# Autodesk Inventor assembly: Złożenie całości
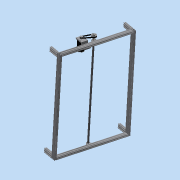
[picture p0: Inventor's stored thumbnail of the model, 180x180]
Saved by Autodesk Inventor 2018 (Build 220112000, 112)
## iProperties
Created: 2019-01-23
Part Number: Złożenie całości
Material: Ogólny
Document SubType Name: Assembly
Designer: Dawid
Author: Dawid
## Documents named in this file (16)
- E:\Frezarka_K2\INVENTOR\ZŁOŻENIA\Złożenie całości.iam
- E:\Frezarka_K2\INVENTOR\RAMA\Profil dolny długi.ipt
- E:\Frezarka_K2\INVENTOR\RAMA\Profil dolny krótki.ipt
- E:\Frezarka_K2\INVENTOR\RAMA\Profil dolny - noga.ipt
- E:\Frezarka_K2\INVENTOR\NAPĘD\Śruba trapezowa 16x4.ipt
- E:\Frezarka_K2\INVENTOR\NAPĘD\Łożysko w obudowie aluminiowej 10mm KP000.ipt
- C:\Users\Dawid\Documents\Inventor\Content Center Files\R2018\pl-PL\DIN 6926\DIN 6926 - M10 x 1,5.ipt
- E:\Frezarka_K2\INVENTOR\NAPĘD\Koło zębate 21 T5 28 2F.ipt
- E:\Frezarka_K2\INVENTOR\NAPĘD\Tuleja zaciskowo rozprężna RCK BK 80 8x15 Clampex.ipt
- C:\Users\Dawid\Documents\Inventor\Content Center Files\R2018\pl-PL\CNS 3932\CNS 3932 - M 4 x 0,7 x 6.ipt
- E:\Frezarka_K2\INVENTOR\NAPĘD\Silnik krokowy SM 60 100-4004AF - 4Nm.ipt
- E:\Frezarka_K2\INVENTOR\NAPĘD\Koło zębate 21 T5 14 2F.ipt
- E:\Frezarka_K2\INVENTOR\NAPĘD\Uchwyt silnika krokowego osi Y.ipt
- C:\Users\Dawid\Documents\Inventor\Content Center Files\R2018\pl-PL\CNS 3932\CNS 3932 - M 5 x 0,8 x 12.ipt
- E:\Frezarka_K2\INVENTOR\NAPĘD\Pas zębaty 10 T5-315.ipt
- C:\Users\Dawid\Documents\Inventor\Content Center Files\R2018\pl-PL\CNS 3932\CNS 3932 - M 5 x 0,8 x 10.ipt
## Components (32 placed, 15 different names)
1. Profil dolny długi:1 — Zestawiający:1, Równoległy:1, Równoległy:2, Zestawiający:4, Równoległy:7, Zestawiający:7, Równoległy:13, Równoległy:14
2. Profil dolny krótki:1 — Zestawiający:1, Równoległy:1, Równoległy:2, Zestawiający:2, Równoległy:3, Równoległy:4, Zestawiający:15
3. Profil dolny długi:2 — Zestawiający:2, Równoległy:3, Równoległy:4, Zestawiający:3, Równoległy:5, Zestawiający:5, Równoległy:9, Równoległy:10, Zestawiający:6, Równoległy:11, Równoległy:12, Równoległy:15, Zestawiający:20
4. Profil dolny krótki:2 — Zestawiający:3, Równoległy:5, Równoległy:8, Równoległy:15, Zestawiający:14, Równoległy:16, Zestawiający:26, Zestawiający:27, Zestawiający:30
5. Profil dolny - noga:1 — Zestawiający:5, Równoległy:9, Równoległy:10
6. Profil dolny - noga:2 — Zestawiający:6, Równoległy:11, Równoległy:12
7. Profil dolny - noga:3 — Zestawiający:7, Równoległy:13, Równoległy:14
8. Profil dolny - noga:4 — Zestawiający:4, Równoległy:7, Równoległy:8
9. Śruba trapezowa 16x4:1 — Zestawiający:8, Zestawiający:9, Zestawiający:10, Zestawiający:11, Zestawiający:12, Zestawiający:18, Zestawiający:19
10. Łożysko w obudowie aluminiowej 10mm KP000:1 — Zestawiający:8, Zestawiający:9, Zestawiający:13, Zestawiający:14, Równoległy:16, Zestawiający:20
11. Łożysko w obudowie aluminiowej 10mm KP000:2 — Zestawiający:10, Zestawiający:11, Zestawiający:15
12. DIN 6926 - zastąpiona przez DIN EN 1663/1666 M10:1 — Zestawiający:12, Zestawiający:13
13. Koło zębate 21 T5 28 2F:1 — Zestawiający:16, Zestawiający:17, Zestawiający:28
14. Tuleja zaciskowo rozprężna RCK BK 80 8x15 Clampex:1 — Zestawiający:16, Zestawiający:17, Zestawiający:18, Zestawiający:19, Wstaw:1, Wstaw:2, Wstaw:3, Wstaw:4, Wstaw:5, Wstaw:6
15. CNS 3932 M 4 x 6:1 — Wstaw:1
16. CNS 3932 M 4 x 6:2 — Wstaw:2
17. CNS 3932 M 4 x 6:3 — Wstaw:3
18. CNS 3932 M 4 x 6:4 — Wstaw:4
19. CNS 3932 M 4 x 6:5 — Wstaw:5
20. CNS 3932 M 4 x 6:6 — Wstaw:6
21. Silnik krokowy SM 60 100-4004AF - 4Nm:1 — Zestawiający:21, Zestawiający:22, Zestawiający:23, Zestawiający:24, Zestawiający:25, Wstaw:7, Wstaw:8, Wstaw:9, Wstaw:10
22. Koło zębate 21 T5 14 2F:1 — Zestawiający:21, Zestawiający:22, Zestawiający:27, Zestawiający:29
23. Uchwyt silnika krokowego osi Y:1 — Zestawiający:23, Zestawiający:24, Zestawiający:25, Zestawiający:26, Zestawiający:30, Wstaw:11, Wstaw:12, Wstaw:13, Wstaw:14
24. CNS 3932 M 5 x 12:1 — Wstaw:7
25. CNS 3932 M 5 x 12:2 — Wstaw:8
26. CNS 3932 M 5 x 12:3 — Wstaw:9
27. CNS 3932 M 5 x 12:4 — Wstaw:10
28. Pas zębaty 10 T5-315:1 — Zestawiający:28, Zestawiający:29
29. CNS 3932 M 5 x 10:1 — Wstaw:11
30. CNS 3932 M 5 x 10:2 — Wstaw:12
31. CNS 3932 M 5 x 10:3 — Wstaw:13
32. CNS 3932 M 5 x 10:4 — Wstaw:14
## Relationships (59: Mate 30, Flush 15, Insert 14)
- Zestawiający:1 [Mate]: Profil dolny długi:1 ↔ Profil dolny krótki:1
- Równoległy:1 [Flush]: Profil dolny długi:1 ↔ Profil dolny krótki:1
- Równoległy:2 [Flush]: Profil dolny długi:1 ↔ Profil dolny krótki:1
- Zestawiający:2 [Mate]: Profil dolny krótki:1 ↔ Profil dolny długi:2
- Równoległy:3 [Flush]: Profil dolny krótki:1 ↔ Profil dolny długi:2
- Równoległy:4 [Flush]: Profil dolny krótki:1 ↔ Profil dolny długi:2
- Zestawiający:3 [Mate]: Profil dolny długi:2 ↔ Profil dolny krótki:2
- Równoległy:5 [Flush]: Profil dolny długi:2 ↔ Profil dolny krótki:2
- Zestawiający:4 [Mate]: Profil dolny długi:1 ↔ Profil dolny - noga:4
- Równoległy:7 [Flush]: Profil dolny długi:1 ↔ Profil dolny - noga:4
- Równoległy:8 [Flush]: Profil dolny krótki:2 ↔ Profil dolny - noga:4
- Zestawiający:5 [Mate]: Profil dolny długi:2 ↔ Profil dolny - noga:1
- Równoległy:9 [Flush]: Profil dolny długi:2 ↔ Profil dolny - noga:1
- Równoległy:10 [Flush]: Profil dolny długi:2 ↔ Profil dolny - noga:1
- Zestawiający:6 [Mate]: Profil dolny długi:2 ↔ Profil dolny - noga:2
- Równoległy:11 [Flush]: Profil dolny długi:2 ↔ Profil dolny - noga:2
- Równoległy:12 [Flush]: Profil dolny długi:2 ↔ Profil dolny - noga:2
- Zestawiający:7 [Mate]: Profil dolny długi:1 ↔ Profil dolny - noga:3
- Równoległy:13 [Flush]: Profil dolny długi:1 ↔ Profil dolny - noga:3
- Równoległy:14 [Flush]: Profil dolny długi:1 ↔ Profil dolny - noga:3
- Zestawiający:8 [Mate]: Śruba trapezowa 16x4:1 ↔ Łożysko w obudowie aluminiowej 10mm KP000:1
- Zestawiający:9 [Mate]: Śruba trapezowa 16x4:1 ↔ Łożysko w obudowie aluminiowej 10mm KP000:1
- Zestawiający:10 [Mate]: Śruba trapezowa 16x4:1 ↔ Łożysko w obudowie aluminiowej 10mm KP000:2
- Zestawiający:11 [Mate] (2 mm): Śruba trapezowa 16x4:1 ↔ Łożysko w obudowie aluminiowej 10mm KP000:2
- Zestawiający:12 [Mate]: Śruba trapezowa 16x4:1 ↔ DIN 6926 - zastąpiona przez DIN EN 1663/1666 M10:1
- Zestawiający:13 [Mate]: Łożysko w obudowie aluminiowej 10mm KP000:1 ↔ DIN 6926 - zastąpiona przez DIN EN 1663/1666 M10:1
- Równoległy:15 [Flush]: Profil dolny długi:2 ↔ Profil dolny krótki:2
- Zestawiający:14 [Mate]: Profil dolny krótki:2 ↔ Łożysko w obudowie aluminiowej 10mm KP000:1
- Równoległy:16 [Flush] (2 mm): Profil dolny krótki:2 ↔ Łożysko w obudowie aluminiowej 10mm KP000:1
- Zestawiający:15 [Mate]: Profil dolny krótki:1 ↔ Łożysko w obudowie aluminiowej 10mm KP000:2
- Zestawiający:16 [Mate]: Koło zębate 21 T5 28 2F:1 ↔ Tuleja zaciskowo rozprężna RCK BK 80 8x15 Clampex:1
- Zestawiający:17 [Mate]: Koło zębate 21 T5 28 2F:1 ↔ Tuleja zaciskowo rozprężna RCK BK 80 8x15 Clampex:1
- Zestawiający:18 [Mate]: Śruba trapezowa 16x4:1 ↔ Tuleja zaciskowo rozprężna RCK BK 80 8x15 Clampex:1
- Zestawiający:19 [Mate] (2 mm): Śruba trapezowa 16x4:1 ↔ Tuleja zaciskowo rozprężna RCK BK 80 8x15 Clampex:1
- Wstaw:1 [Insert]: Tuleja zaciskowo rozprężna RCK BK 80 8x15 Clampex:1 ↔ CNS 3932 M 4 x 6:1
- Wstaw:2 [Insert]: Tuleja zaciskowo rozprężna RCK BK 80 8x15 Clampex:1 ↔ CNS 3932 M 4 x 6:2
- Wstaw:3 [Insert]: Tuleja zaciskowo rozprężna RCK BK 80 8x15 Clampex:1 ↔ CNS 3932 M 4 x 6:3
- Wstaw:4 [Insert]: Tuleja zaciskowo rozprężna RCK BK 80 8x15 Clampex:1 ↔ CNS 3932 M 4 x 6:4
- Wstaw:5 [Insert]: Tuleja zaciskowo rozprężna RCK BK 80 8x15 Clampex:1 ↔ CNS 3932 M 4 x 6:5
- Wstaw:6 [Insert]: Tuleja zaciskowo rozprężna RCK BK 80 8x15 Clampex:1 ↔ CNS 3932 M 4 x 6:6
- Zestawiający:20 [Mate] (296.5 mm): Profil dolny długi:2 ↔ Łożysko w obudowie aluminiowej 10mm KP000:1
- Zestawiający:21 [Mate]: Silnik krokowy SM 60 100-4004AF - 4Nm:1 ↔ Koło zębate 21 T5 14 2F:1
- Zestawiający:22 [Mate] (1 mm): Silnik krokowy SM 60 100-4004AF - 4Nm:1 ↔ Koło zębate 21 T5 14 2F:1
- Zestawiający:23 [Mate]: Silnik krokowy SM 60 100-4004AF - 4Nm:1 ↔ Uchwyt silnika krokowego osi Y:1
- Zestawiający:24 [Mate]: Silnik krokowy SM 60 100-4004AF - 4Nm:1 ↔ Uchwyt silnika krokowego osi Y:1
- Zestawiający:25 [Mate]: Silnik krokowy SM 60 100-4004AF - 4Nm:1 ↔ Uchwyt silnika krokowego osi Y:1
- Zestawiający:26 [Mate]: Profil dolny krótki:2 ↔ Uchwyt silnika krokowego osi Y:1
- Zestawiający:27 [Mate] (40 mm): Profil dolny krótki:2 ↔ Koło zębate 21 T5 14 2F:1
- Wstaw:7 [Insert]: Silnik krokowy SM 60 100-4004AF - 4Nm:1 ↔ CNS 3932 M 5 x 12:1
- Wstaw:8 [Insert]: Silnik krokowy SM 60 100-4004AF - 4Nm:1 ↔ CNS 3932 M 5 x 12:2
- Wstaw:9 [Insert]: Silnik krokowy SM 60 100-4004AF - 4Nm:1 ↔ CNS 3932 M 5 x 12:3
- Wstaw:10 [Insert]: Silnik krokowy SM 60 100-4004AF - 4Nm:1 ↔ CNS 3932 M 5 x 12:4
- Zestawiający:28 [Mate]: Koło zębate 21 T5 28 2F:1 ↔ Pas zębaty 10 T5-315:1
- Zestawiający:29 [Mate]: Koło zębate 21 T5 14 2F:1 ↔ Pas zębaty 10 T5-315:1
- Zestawiający:30 [Mate]: Profil dolny krótki:2 ↔ Uchwyt silnika krokowego osi Y:1
- Wstaw:11 [Insert]: Uchwyt silnika krokowego osi Y:1 ↔ CNS 3932 M 5 x 10:1
- Wstaw:12 [Insert]: Uchwyt silnika krokowego osi Y:1 ↔ CNS 3932 M 5 x 10:2
- Wstaw:13 [Insert]: Uchwyt silnika krokowego osi Y:1 ↔ CNS 3932 M 5 x 10:3
- Wstaw:14 [Insert]: Uchwyt silnika krokowego osi Y:1 ↔ CNS 3932 M 5 x 10:4
